# Autodesk Inventor assembly: Assembly_FINAL
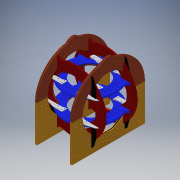
[picture p0: Inventor's stored thumbnail of the model, 180x180]
Saved by Autodesk Inventor 2016 (Build 200138000, 138)
## iProperties
Created: 2016-01-31
Part Number: Assembly_FINAL
Document SubType Name: Assembly
Designer: Scott
Author: Scott
## Documents named in this file (10)
- C:\Users\Matt\Documents\BTSync\CubeSat\Cleaned_Up_Helmholtz_Model_for_Manual\Parts\Assembly_FINAL.iam
- C:\Users\Matt\Documents\BTSync\CubeSat\Cleaned_Up_Helmholtz_Model_for_Manual\Parts\Large_Coil_Inner.ipt
- C:\Users\Matt\Documents\BTSync\CubeSat\Cleaned_Up_Helmholtz_Model_for_Manual\Parts\Large_Coil_Outer_Bottom.ipt
- C:\Users\Matt\Documents\BTSync\CubeSat\Cleaned_Up_Helmholtz_Model_for_Manual\Parts\Medium_Coil_Inner.ipt
- C:\Users\Matt\Documents\BTSync\CubeSat\Cleaned_Up_Helmholtz_Model_for_Manual\Parts\Medium_Coil_Outer.ipt
- C:\Users\Matt\Documents\BTSync\CubeSat\Cleaned_Up_Helmholtz_Model_for_Manual\Parts\Small_Coil_Inner.ipt
- C:\Users\Matt\Documents\BTSync\CubeSat\Cleaned_Up_Helmholtz_Model_for_Manual\Parts\Small_Coil_Outer.ipt
- C:\Users\Matt\Documents\BTSync\CubeSat\Cleaned_Up_Helmholtz_Model_for_Manual\Parts\Outer_Coil_Retainer.ipt
- C:\Users\Matt\Documents\BTSync\CubeSat\Cleaned_Up_Helmholtz_Model_for_Manual\Parts\Inner_Coil_Retainer.ipt
- C:\Users\Matt\Documents\BTSync\CubeSat\Cleaned_Up_Helmholtz_Model_for_Manual\Parts\Large_Coil_Outer_Top.ipt
## Components (52 placed, 9 different names)
1. Large_Coil_Inner:1 — Mate:1, Mate:2, Flush:1, Mate:3, Mate:9, Mate:174
2. Large_Coil_Inner:2 — Mate:1, Mate:2, Flush:1, Mate:4, Mate:5, Mate:10, Mate:175, Mate:180, Mate:181
3. Large_Coil_Outer_Bottom:1 — Mate:9, Flush:2, Mate:10, Flush:10, Mate:112, Mate:136, Mate:176
4. Large_Coil_Outer_Bottom:2 — Mate:3, Mate:4, Mate:5, Flush:2, Flush:5, Flush:6, Mate:182
5. Large_Coil_Inner:3
6. Large_Coil_Inner:4 — Mate:177, Mate:178, Mate:183, Mate:184
7. Large_Coil_Outer_Bottom:3 — Flush:5, Flush:6, Mate:179
8. Large_Coil_Outer_Bottom:4 — Mate:97, Mate:107, Mate:185
9. Medium_Coil_Inner:1 — Flush:7, Mate:29, Mate:30, Mate:47, Mate:49, Mate:51, Mate:52, Mate:58
10. Medium_Coil_Inner:2 — Flush:7, Mate:29, Mate:30, Mate:48, Mate:50, Mate:53, Mate:55, Mate:56
11. Medium_Coil_Inner:3 — Mate:27, Mate:28, Flush:8, Mate:37, Mate:39, Mate:40, Mate:41, Mate:43, Mate:44, Mate:61
12. Medium_Coil_Inner:4 — Mate:27, Mate:28, Flush:8, Mate:32, Mate:42
13. Medium_Coil_Outer:1 — Mate:35, Mate:37, Mate:38, Mate:59, Mate:62
14. Medium_Coil_Outer:2 — Mate:32, Mate:35, Mate:38, Mate:39, Mate:40
15. Medium_Coil_Outer:3 — Mate:41, Mate:42, Mate:43, Mate:92, Mate:95, Symmetry:2, Mate:137, Mate:139, Mate:140, Mate:152
16. Medium_Coil_Outer:4 — Mate:44, Flush:10, Mate:91, Mate:96, Mate:137, Mate:166
17. Medium_Coil_Outer:5 — Mate:47, Mate:48, Mate:49, Mate:54
18. Medium_Coil_Outer:6 — Mate:50, Mate:51, Mate:52, Mate:62, Mate:135
19. Medium_Coil_Outer:7 — Mate:56, Mate:57, Mate:58, Mate:104, Mate:106, Mate:131, Mate:143, Mate:144, Mate:168, Mate:171
20. Medium_Coil_Outer:8 — Mate:53, Mate:54, Mate:55, Mate:57, Mate:59, Mate:61, Mate:103, Mate:105, Symmetry:2, Mate:141, Mate:142, Mate:153
21. Small_Coil_Inner:1 — Flush:11, Mate:77, Mate:78, Mate:81, Mate:84, Mate:86, Mate:89
22. Small_Coil_Outer:1 — Mate:85, Mate:86, Mate:87
23. Outer_Coil_Retainer:1 — Mate:91, Mate:136
24. Small_Coil_Inner:2 — Flush:11, Mate:77, Mate:78, Mate:79, Mate:80, Mate:82, Mate:83, Mate:85, Mate:87, Mate:88, Mate:90, Mate:129
25. Small_Coil_Outer:2 — Mate:79, Mate:80, Mate:81, Mate:130, Flush:13, Mate:162, Mate:163, Mate:167, Mate:169
26. Outer_Coil_Retainer:2 — Mate:92, Mate:140
27. Small_Coil_Outer:3 — Mate:82, Mate:83, Mate:84, Mate:134, Mate:161, Mate:164, Mate:165, Mate:170
28. Outer_Coil_Retainer:3 — Mate:106, Mate:107, Mate:144
29. Small_Coil_Outer:4 — Mate:88, Mate:89, Mate:90
30. Outer_Coil_Retainer:4 — Mate:96, Mate:97
31. Outer_Coil_Retainer:5 — Mate:95, Mate:139
32. Outer_Coil_Retainer:6 — Mate:103, Mate:141
33. Outer_Coil_Retainer:7 — Mate:104, Mate:112, Mate:143
34. Outer_Coil_Retainer:8 — Mate:105, Mate:142
35. Small_Coil_Inner:3
36. Small_Coil_Outer:5
37. Small_Coil_Inner:4 — Mate:129, Mate:133, Mate:149
38. Small_Coil_Outer:6 — Flush:13, Mate:158, Mate:159, Mate:160
39. Small_Coil_Outer:7 — Mate:132, Mate:148, Mate:150, Mate:151, Mate:154, Mate:155, Mate:156, Mate:157
40. Small_Coil_Outer:8 — Mate:130, Mate:131, Mate:149
41. Inner_Coil_Retainer:1 — Mate:155, Mate:156, Mate:157
42. Inner_Coil_Retainer:2 — Mate:151, Mate:152, Mate:158
43. Inner_Coil_Retainer:4 — Mate:148, Mate:153, Mate:154
44. Inner_Coil_Retainer:5 — Mate:150, Mate:159, Mate:160
45. Inner_Coil_Retainer:6 — Mate:161, Mate:164, Mate:165
46. Inner_Coil_Retainer:7 — Flush:14, Mate:163, Mate:166, Mate:167
47. Inner_Coil_Retainer:8 — Mate:162, Mate:168, Mate:169
48. Inner_Coil_Retainer:9 — Flush:14, Mate:170, Mate:171
49. Large_Coil_Outer_Top:1 — Mate:174, Mate:175, Mate:176
50. Large_Coil_Outer_Top:2 — Mate:177, Mate:178, Mate:179
51. Large_Coil_Outer_Top:3 — Mate:180, Mate:181, Mate:182
52. Large_Coil_Outer_Top:4 — Mate:183, Mate:184, Mate:185
## Relationships (147: Mate 133, Flush 13, Symmetry 1)
- Mate:1: Large_Coil_Inner:1 ↔ Large_Coil_Inner:2
- Mate:2: Large_Coil_Inner:1 ↔ Large_Coil_Inner:2
- Flush:1: Large_Coil_Inner:1 ↔ Large_Coil_Inner:2
- Mate:3: Large_Coil_Inner:1 ↔ Large_Coil_Outer_Bottom:2
- Mate:4: Large_Coil_Inner:2 ↔ Large_Coil_Outer_Bottom:2
- Mate:5: Large_Coil_Inner:2 ↔ Large_Coil_Outer_Bottom:2
- Mate:9: Large_Coil_Inner:1 ↔ Large_Coil_Outer_Bottom:1
- Flush:2: Large_Coil_Outer_Bottom:1 ↔ Large_Coil_Outer_Bottom:2
- Mate:10: Large_Coil_Inner:2 ↔ Large_Coil_Outer_Bottom:1
- [Mate]: Large_Coil_Inner:3 ↔ Large_Coil_Inner:4
- [Mate]: Large_Coil_Inner:3 ↔ Large_Coil_Inner:4
- [Flush]: Large_Coil_Inner:3 ↔ Large_Coil_Inner:4
- [Mate]: Large_Coil_Inner:3 ↔ Large_Coil_Outer_Bottom:4
- [Mate]: Large_Coil_Inner:4 ↔ Large_Coil_Outer_Bottom:4
- [Mate]: Large_Coil_Inner:4 ↔ Large_Coil_Outer_Bottom:4
- [Mate]: Large_Coil_Inner:3 ↔ Large_Coil_Outer_Bottom:3
- [Flush]: Large_Coil_Outer_Bottom:3 ↔ Large_Coil_Outer_Bottom:4
- [Mate]: Large_Coil_Inner:4 ↔ Large_Coil_Outer_Bottom:3
- Flush:5: Large_Coil_Outer_Bottom:2 ↔ Large_Coil_Outer_Bottom:3
- Flush:6: Large_Coil_Outer_Bottom:2 ↔ Large_Coil_Outer_Bottom:3
- Mate:27: Medium_Coil_Inner:3 ↔ Medium_Coil_Inner:4
- Mate:28: Medium_Coil_Inner:3 ↔ Medium_Coil_Inner:4
- Flush:7: Medium_Coil_Inner:1 ↔ Medium_Coil_Inner:2
- Mate:29: Medium_Coil_Inner:1 ↔ Medium_Coil_Inner:2
- Mate:30: Medium_Coil_Inner:1 ↔ Medium_Coil_Inner:2
- Flush:8: Medium_Coil_Inner:3 ↔ Medium_Coil_Inner:4
- Mate:32: Medium_Coil_Inner:4 ↔ Medium_Coil_Outer:2
- Mate:35: Medium_Coil_Outer:1 ↔ Medium_Coil_Outer:2
- Mate:37: Medium_Coil_Inner:3 ↔ Medium_Coil_Outer:1
- Mate:38: Medium_Coil_Outer:1 ↔ Medium_Coil_Outer:2
- Mate:39: Medium_Coil_Inner:3 ↔ Medium_Coil_Outer:2
- Mate:40: Medium_Coil_Inner:3 ↔ Medium_Coil_Outer:2
- Mate:41: Medium_Coil_Inner:3 ↔ Medium_Coil_Outer:3
- Mate:42: Medium_Coil_Inner:4 ↔ Medium_Coil_Outer:3
- Mate:43: Medium_Coil_Inner:3 ↔ Medium_Coil_Outer:3
- Mate:44: Medium_Coil_Inner:3 ↔ Medium_Coil_Outer:4
- Mate:47: Medium_Coil_Inner:1 ↔ Medium_Coil_Outer:5
- Mate:48: Medium_Coil_Inner:2 ↔ Medium_Coil_Outer:5
- Mate:49: Medium_Coil_Inner:1 ↔ Medium_Coil_Outer:5
- Mate:50: Medium_Coil_Inner:2 ↔ Medium_Coil_Outer:6
- Mate:51: Medium_Coil_Inner:1 ↔ Medium_Coil_Outer:6
- Mate:52: Medium_Coil_Inner:1 ↔ Medium_Coil_Outer:6
- Mate:53: Medium_Coil_Inner:2 ↔ Medium_Coil_Outer:8
- Mate:54: Medium_Coil_Outer:5 ↔ Medium_Coil_Outer:8
- Mate:55: Medium_Coil_Inner:2 ↔ Medium_Coil_Outer:8
- Mate:56: Medium_Coil_Inner:2 ↔ Medium_Coil_Outer:7
- Mate:57: Medium_Coil_Outer:7 ↔ Medium_Coil_Outer:8
- Mate:58: Medium_Coil_Inner:1 ↔ Medium_Coil_Outer:7
- Mate:59: Medium_Coil_Outer:1 ↔ Medium_Coil_Outer:8
- Mate:61: Medium_Coil_Inner:3 ↔ Medium_Coil_Outer:8
- Mate:62 (203.2 mm): Medium_Coil_Outer:1 ↔ Medium_Coil_Outer:6
- Flush:10: Large_Coil_Outer_Bottom:1 ↔ Medium_Coil_Outer:4
- Flush:11: Small_Coil_Inner:1 ↔ Small_Coil_Inner:2
- Mate:77: Small_Coil_Inner:1 ↔ Small_Coil_Inner:2
- Mate:78: Small_Coil_Inner:1 ↔ Small_Coil_Inner:2
- Mate:79: Small_Coil_Inner:2 ↔ Small_Coil_Outer:2
- Mate:80: Small_Coil_Inner:2 ↔ Small_Coil_Outer:2
- Mate:81: Small_Coil_Inner:1 ↔ Small_Coil_Outer:2
- Mate:82: Small_Coil_Inner:2 ↔ Small_Coil_Outer:3
- Mate:83: Small_Coil_Inner:2 ↔ Small_Coil_Outer:3
- Mate:84: Small_Coil_Inner:1 ↔ Small_Coil_Outer:3
- Mate:85: Small_Coil_Outer:1 ↔ Small_Coil_Inner:2
- Mate:86: Small_Coil_Inner:1 ↔ Small_Coil_Outer:1
- Mate:87: Small_Coil_Outer:1 ↔ Small_Coil_Inner:2
- Mate:88: Small_Coil_Inner:2 ↔ Small_Coil_Outer:4
- Mate:89: Small_Coil_Inner:1 ↔ Small_Coil_Outer:4
- Mate:90: Small_Coil_Inner:2 ↔ Small_Coil_Outer:4
- Mate:91: Medium_Coil_Outer:4 ↔ Outer_Coil_Retainer:1
- Mate:92: Medium_Coil_Outer:3 ↔ Outer_Coil_Retainer:2
- Mate:95: Medium_Coil_Outer:3 ↔ Outer_Coil_Retainer:5
- Mate:96: Medium_Coil_Outer:4 ↔ Outer_Coil_Retainer:4
- Mate:97: Large_Coil_Outer_Bottom:4 ↔ Outer_Coil_Retainer:4
- Mate:103: Medium_Coil_Outer:8 ↔ Outer_Coil_Retainer:6
- Mate:104: Medium_Coil_Outer:7 ↔ Outer_Coil_Retainer:7
- Mate:105: Medium_Coil_Outer:8 ↔ Outer_Coil_Retainer:8
- Mate:106: Medium_Coil_Outer:7 ↔ Outer_Coil_Retainer:3
- Mate:107: Large_Coil_Outer_Bottom:4 ↔ Outer_Coil_Retainer:3
- Mate:112: Large_Coil_Outer_Bottom:1 ↔ Outer_Coil_Retainer:7
- [Flush]: Small_Coil_Inner:3 ↔ Small_Coil_Inner:4
- [Mate]: Small_Coil_Inner:3 ↔ Small_Coil_Inner:4
- [Mate]: Small_Coil_Inner:3 ↔ Small_Coil_Inner:4
- [Mate]: Small_Coil_Inner:4 ↔ Small_Coil_Outer:6
- [Mate]: Small_Coil_Inner:4 ↔ Small_Coil_Outer:6
- [Mate]: Small_Coil_Inner:3 ↔ Small_Coil_Outer:6
- [Mate]: Small_Coil_Inner:4 ↔ Small_Coil_Outer:7
- [Mate]: Small_Coil_Inner:4 ↔ Small_Coil_Outer:7
- [Mate]: Small_Coil_Inner:3 ↔ Small_Coil_Outer:7
- [Mate]: Small_Coil_Outer:5 ↔ Small_Coil_Inner:4
- [Mate]: Small_Coil_Inner:3 ↔ Small_Coil_Outer:5
- [Mate]: Small_Coil_Outer:5 ↔ Small_Coil_Inner:4
- [Mate]: Small_Coil_Inner:4 ↔ Small_Coil_Outer:8
- [Mate]: Small_Coil_Inner:3 ↔ Small_Coil_Outer:8
- [Mate]: Small_Coil_Inner:4 ↔ Small_Coil_Outer:8
- Mate:129: Small_Coil_Inner:2 ↔ Small_Coil_Inner:4
- Mate:130 (152.4 mm): Small_Coil_Outer:2 ↔ Small_Coil_Outer:8
- Mate:131 (76.2 mm): Medium_Coil_Outer:7 ↔ Small_Coil_Outer:8
- Mate:132: Small_Coil_Outer:7
- Symmetry:2: Medium_Coil_Outer:3 ↔ Medium_Coil_Outer:8
- Mate:133: Small_Coil_Inner:4
- Mate:134: Small_Coil_Outer:3
- Mate:135: Medium_Coil_Outer:6
- Flush:13: Small_Coil_Outer:2 ↔ Small_Coil_Outer:6
- Mate:136: Large_Coil_Outer_Bottom:1 ↔ Outer_Coil_Retainer:1
- Mate:137: Medium_Coil_Outer:3 ↔ Medium_Coil_Outer:4
- Mate:139: Medium_Coil_Outer:3 ↔ Outer_Coil_Retainer:5
- Mate:140: Medium_Coil_Outer:3 ↔ Outer_Coil_Retainer:2
- Mate:141: Medium_Coil_Outer:8 ↔ Outer_Coil_Retainer:6
- Mate:142: Medium_Coil_Outer:8 ↔ Outer_Coil_Retainer:8
- Mate:143: Medium_Coil_Outer:7 ↔ Outer_Coil_Retainer:7
- Mate:144: Medium_Coil_Outer:7 ↔ Outer_Coil_Retainer:3
- Mate:148: Small_Coil_Outer:7 ↔ Inner_Coil_Retainer:4
- Mate:149: Small_Coil_Inner:4 ↔ Small_Coil_Outer:8
- Mate:150: Small_Coil_Outer:7 ↔ Inner_Coil_Retainer:5
- Mate:151: Small_Coil_Outer:7 ↔ Inner_Coil_Retainer:2
- Mate:152: Medium_Coil_Outer:3 ↔ Inner_Coil_Retainer:2
- Mate:153: Medium_Coil_Outer:8 ↔ Inner_Coil_Retainer:4
- Mate:154: Small_Coil_Outer:7 ↔ Inner_Coil_Retainer:4
- Mate:155: Small_Coil_Outer:7 ↔ Inner_Coil_Retainer:1
- Mate:156: Small_Coil_Outer:7 ↔ Inner_Coil_Retainer:1
- Mate:157: Small_Coil_Outer:7 ↔ Inner_Coil_Retainer:1
- Mate:158: Small_Coil_Outer:6 ↔ Inner_Coil_Retainer:2
- Mate:159: Small_Coil_Outer:6 ↔ Inner_Coil_Retainer:5
- Mate:160: Small_Coil_Outer:6 ↔ Inner_Coil_Retainer:5
- Mate:161: Small_Coil_Outer:3 ↔ Inner_Coil_Retainer:6
- Mate:162: Small_Coil_Outer:2 ↔ Inner_Coil_Retainer:8
- Flush:14: Inner_Coil_Retainer:7 ↔ Inner_Coil_Retainer:9
- Mate:163: Small_Coil_Outer:2 ↔ Inner_Coil_Retainer:7
- Mate:164: Small_Coil_Outer:3 ↔ Inner_Coil_Retainer:6
- Mate:165: Small_Coil_Outer:3 ↔ Inner_Coil_Retainer:6
- Mate:166: Medium_Coil_Outer:4 ↔ Inner_Coil_Retainer:7
- Mate:167: Small_Coil_Outer:2 ↔ Inner_Coil_Retainer:7
- Mate:168: Medium_Coil_Outer:7 ↔ Inner_Coil_Retainer:8
- Mate:169: Small_Coil_Outer:2 ↔ Inner_Coil_Retainer:8
- Mate:170: Small_Coil_Outer:3 ↔ Inner_Coil_Retainer:9
- Mate:171: Medium_Coil_Outer:7 ↔ Inner_Coil_Retainer:9
- Mate:174: Large_Coil_Inner:1 ↔ Large_Coil_Outer_Top:1
- Mate:175: Large_Coil_Inner:2 ↔ Large_Coil_Outer_Top:1
- Mate:176: Large_Coil_Outer_Bottom:1 ↔ Large_Coil_Outer_Top:1
- Mate:177: Large_Coil_Inner:4 ↔ Large_Coil_Outer_Top:2
- Mate:178: Large_Coil_Inner:4 ↔ Large_Coil_Outer_Top:2
- Mate:179: Large_Coil_Outer_Bottom:3 ↔ Large_Coil_Outer_Top:2
- Mate:180: Large_Coil_Inner:2 ↔ Large_Coil_Outer_Top:3
- Mate:181: Large_Coil_Inner:2 ↔ Large_Coil_Outer_Top:3
- Mate:182: Large_Coil_Outer_Bottom:2 ↔ Large_Coil_Outer_Top:3
- Mate:183: Large_Coil_Inner:4 ↔ Large_Coil_Outer_Top:4
- Mate:184: Large_Coil_Inner:4 ↔ Large_Coil_Outer_Top:4
- Mate:185: Large_Coil_Outer_Bottom:4 ↔ Large_Coil_Outer_Top:4
## Named parameters: d16_d4 = 0 mm, d17_d5 = 0 mm, d18_d6 = 0 mm, d22_d10 = 0 mm, d23_d11 = 0 mm, d24_d12 = 0 mm, d28_d2 = 0 mm, d29_d0 = 0 mm, d30_d1 = 0 mm, d132_d93 = 0 mm, d133_d94 = 0 mm, d134_d95 = 0 mm, d135_d96 = 0 mm, d136_d97 = 0 mm, d137_d98 = 0 mm, d138_d99 = 0 mm, d139_d100 = 0 mm, d140_d101 = 0 mm, d141_d102 = 0 mm, d142_d103 = 0 mm, d143_d104 = 0 mm, d144_d105 = 0 mm, d145_d106 = 0 mm, d146_d107 = 0 mm
